# Autodesk Inventor assembly: landing_gear
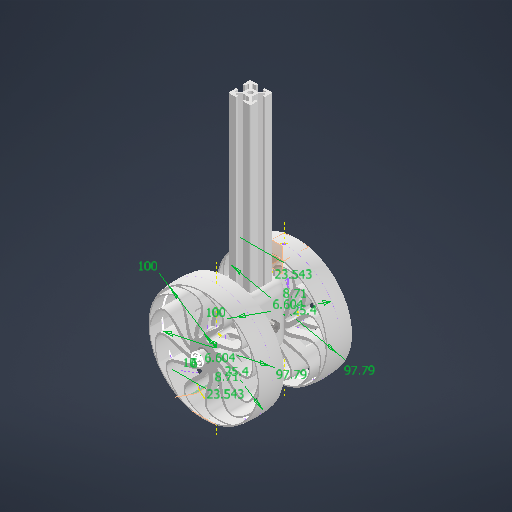
[picture p0: Inventor's stored thumbnail of the model, 512x512]
Saved by Autodesk Inventor 2027 (Build 310192060, 192F)
## iProperties
Created: 2026-06-22
Part Number: landing_gear
Document SubType Name: Assembly
Designer: localadmin
Author: localadmin
## Documents named in this file (9)
- C:\Users\efloy\github\SWIFT-UAV\System_development\Pelican\structural_model\v0.3.0\Parts\LandingGear\landing_gear.iam
- C:\Users\efloy\github\SWIFT-UAV\System_development\Pelican\structural_model\v0.3.0\Parts\LandingGear\arm_collar.ipt
- C:\Users\efloy\OneDrive\Documents\Inventor\Content Center Files\R2027\en-US\ISO 7089\ISO 7089 - 6 - 140 HV(1).ipt
- C:\Users\efloy\github\SWIFT-UAV\System_development\Pelican\structural_model\v0.3.0\Parts\LandingGear\m5_t_nut.ipt
- C:\Users\efloy\OneDrive\Documents\Inventor\Content Center Files\R2027\en-US\ISO 4762(2)\ISO 4762 - M5 x 12ISO.ipt
- C:\Users\efloy\github\SWIFT-UAV\System_development\Pelican\structural_model\v0.3.0\Parts\LandingGear\m6_bolt100mm.ipt
- C:\Users\efloy\OneDrive\Documents\Inventor\Content Center Files\R2027\en-US\ISO 4032(2)\ISO 4032 - M6 - ISO.ipt
- C:\Users\efloy\github\SWIFT-UAV\System_development\Pelican\structural_model\v0.3.0\Parts\LandingGear\20x20alumnium.ipt
- C:\Users\efloy\github\SWIFT-UAV\System_development\Pelican\structural_model\v0.3.0\Parts\LandingGear\12spoke_wheel_final.ipt
## Components (16 placed, 8 different names)
1. arm_collar:1 — Insert:1, Mate:9, Mate:12, Insert:7, Rigid:1
2. ISO 7089 6:1 — Insert:7
3. ISO 7089 6:2 — Insert:11
4. ISO 7089 6:3 — Insert:1, Insert:4
5. ISO 7089 6:4 — Insert:4, Insert:13
6. ISO 7089 6:5 — Insert:14
7. ISO 7089 6:6 — Insert:12
8. m5_t_nut:1 — Mate:9
9. m5_t_nut:2 — Mate:12
10. ISO 4762 M5 x 12:3
11. ISO 4762 M5 x 12:4
12. m6_bolt100mm:1 — Insert:11
13. ISO 4032 M6:1 — Insert:12
14. 20x20alumnium:1 — Rigid:1
15. 12spoke_wheel:1 — Insert:13
16. 12spoke_wheel:2 — Insert:14
## Relationships (10: Insert 7, Mate 2, WeldJoint 1)
- Insert:1: arm_collar:1 ↔ ISO 7089 6:3
- Insert:4: ISO 7089 6:3 ↔ ISO 7089 6:4
- Mate:9: arm_collar:1 ↔ m5_t_nut:1
- Mate:12: arm_collar:1 ↔ m5_t_nut:2
- Insert:7: arm_collar:1 ↔ ISO 7089 6:1
- Insert:11: ISO 7089 6:2 ↔ m6_bolt100mm:1
- Insert:12: ISO 7089 6:6 ↔ ISO 4032 M6:1
- Rigid:1 [WeldJoint]: arm_collar:1 ↔ 20x20alumnium:1
- Insert:13: ISO 7089 6:4 ↔ 12spoke_wheel:1
- Insert:14: ISO 7089 6:5 ↔ 12spoke_wheel:2
